# Autodesk Inventor assembly: base frame
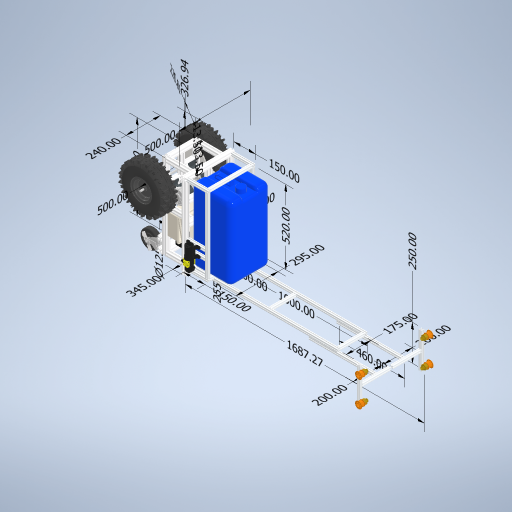
[picture p0: Inventor's stored thumbnail of the model, 512x512]
Saved by Autodesk Inventor 2023 (Build 270158000, 158)
## iProperties
Created: 2023-09-20
Part Number: base frame
Document SubType Name: Assembly
Designer: sigit
Author: sigit
## Documents named in this file (29)
- D:\Kuliah\SEMESTER 7\Robot Semprot\Design\2nd ROBOT\Assembly\base frame.iam
- D:\Kuliah\SEMESTER 7\Robot Semprot\Design\2nd ROBOT\Part\3030 600.ipt
- D:\Kuliah\SEMESTER 7\Robot Semprot\Design\2nd ROBOT\Part\3030 180.ipt
- D:\Kuliah\SEMESTER 7\Robot Semprot\Design\2nd ROBOT\Part\shaft holder 12.ipt
- D:\Kuliah\SEMESTER 7\Robot Semprot\Design\2nd ROBOT\Assembly\roda.iam
- D:\Kuliah\SEMESTER 7\Robot Semprot\Design\2nd ROBOT\Part\poros.ipt
- D:\Kuliah\SEMESTER 7\Robot Semprot\Design\2nd ROBOT\Part\free wheel 5 inch.iam
- D:\Kuliah\SEMESTER 7\Robot Semprot\Design\2nd ROBOT\Part\3030 240.ipt
- D:\Kuliah\SEMESTER 7\Robot Semprot\Design\2nd ROBOT\Part\3030 540.ipt
- D:\Kuliah\SEMESTER 7\Robot Semprot\Design\2nd ROBOT\Part\3030 75.ipt
- D:\Kuliah\SEMESTER 7\Robot Semprot\Design\2nd ROBOT\Assembly\motor+tatakan.iam
- D:\Kuliah\SEMESTER 7\Robot Semprot\Design\2nd ROBOT\Part\3030 800.ipt
- D:\Kuliah\SEMESTER 7\Robot Semprot\Design\2nd ROBOT\Part\3030 440.ipt
- D:\Kuliah\SEMESTER 7\Robot Semprot\Design\2nd ROBOT\Part\3030 470.ipt
- D:\Kuliah\SEMESTER 7\Robot Semprot\Design\2nd ROBOT\Part\jerigenn30L.ipt
- D:\Kuliah\SEMESTER 7\Robot Semprot\Design\2nd ROBOT\Part\3030 160.ipt
- D:\Kuliah\SEMESTER 7\Robot Semprot\Design\2nd ROBOT\Assembly\wadah_jerrycan.iam
- D:\Kuliah\SEMESTER 7\Robot Semprot\Design\2nd ROBOT\Part\3030 285.ipt
- D:\Kuliah\SEMESTER 7\Robot Semprot\Design\2nd ROBOT\Part\3030 113.5.ipt
- D:\Kuliah\SEMESTER 7\Robot Semprot\Design\2nd ROBOT\Part\2020 130.ipt
- D:\Kuliah\SEMESTER 7\Robot Semprot\Design\REVISI2\Part\pompa\bomba good pump.ipt
- D:\Kuliah\SEMESTER 7\Robot Semprot\Design\2nd ROBOT\Part\2020 1000.ipt
- D:\Kuliah\SEMESTER 7\Robot Semprot\Design\2nd ROBOT\Part\2020 460.ipt
- D:\Kuliah\SEMESTER 7\Robot Semprot\Design\2nd ROBOT\Part\2020 200.ipt
- D:\Kuliah\SEMESTER 7\Robot Semprot\Design\2nd ROBOT\Part\2020 250.ipt
- D:\Kuliah\SEMESTER 7\Robot Semprot\Design\2nd ROBOT\Part\2020 175.ipt
- D:\Kuliah\SEMESTER 7\Robot Semprot\Design\2nd ROBOT\Part\Junction Box Assembly.iam
- D:\Kuliah\SEMESTER 7\Robot Semprot\Design\REVISI2\Part\aki\Assembly Inventor\Aki GS GTZ5S.iam
- D:\Kuliah\SEMESTER 7\Robot Semprot\Design\REVISI2\Assembly\nozz.iam
## Components (68 placed, 28 different names)
1. 3030 600:1 — Rotational:1, Rotational:2, Rotational:9, Rotational:10, Rotational:14, Rotational:16, Rotational:18
2. 3030 600:2 — Rotational:3, Rotational:4, Rotational:11, Rotational:17, Rotational:23, Rotational:24
3. 3030 180:1 — Rotational:1, Rotational:3, Rotational:15
4. 3030 180:2 — Rotational:2
5. roda:1 [sub-assembly] — Rotational:6
6. poros:1 — Rotational:5
7. roda:2 [sub-assembly] — Rotational:7
8. free wheel 5 inch:1 [sub-assembly] — Rigid:1
9. free wheel 5 inch:2 [sub-assembly] — Rigid:2
10. 3030 180:4 — Rotational:9
11. 3030 180:5 — Rotational:10
12. 3030 180:6 — Rotational:14
13. 3030 540:1 — Rotational:15, Rotational:19, Rotational:38
14. 3030 75:1 — Rotational:16
15. 3030 75:2 — Rotational:17
16. motor+tatakan:1 [sub-assembly] — Rotational:18
17. motor+tatakan:2 [sub-assembly] — Rotational:19
18. jerigenn30L:1 — Rigid:3
19. wadah_jerrycan:1 [sub-assembly] — Rotational:25, Rotational:28, Rotational:31
20. jerigenn30L:2 — Rigid:4
21. bomba good pump:1 — Rotational:29
22. bomba good pump:2 — Rotational:30
23. 2020 200:1 — Rotational:33, Rotational:35
24. 2020 200:2 — Rotational:34, Rotational:36
25. 2020 250:1 — Rotational:35, Rigid:7
26. 2020 250:2 — Rotational:36, Rigid:6
27. Junction Box Assembly:1 [sub-assembly] — Rigid:5
28. Aki GS GTZ5S:1 [sub-assembly] — Rotational:38, Rigid:5
29. shaft holder 12:1 — Rotational:4, Rotational:5, Rotational:7
30. shaft holder 12:2 — Rotational:6
31. 3030 240:1 — Rotational:11, Rigid:1, Rigid:2
32. 3030 240:2
33. 3030 800:1 — Rotational:21
34. 3030 800:2
35. 3030 470:1 — Rotational:22
36. 3030 470:2
37. 3030 160:5 — Rotational:24, Rotational:26
38. 3030 160:6
39. 3030 285:2 — Rotational:26, Rigid:4
40. 3030 285:3 — Rotational:27
41. 3030 113.5:1 — Rotational:27
42. 3030 113.5:2
43. 2020 460:1 — Rotational:32, Rotational:33
44. 2020 1000:1 — Rotational:31, Rotational:32
45. 2020 460:2 — Rotational:34
46. 2020 1000:2 — Rotational:37
47. 2020 175:1 — Rotational:37
48. 2020 175:2
49. nozz:2 [sub-assembly] — Rigid:7
50. nozz:3 [sub-assembly]
51. nozz:4 [sub-assembly]
52. nozz:5 [sub-assembly]
53. nozz:1 [sub-assembly] — Rigid:6
54. nozz:6 [sub-assembly]
55. nozz:7 [sub-assembly]
56. nozz:8 [sub-assembly]
57. 3030 440:1 — Rotational:21
58. 3030 440:2
59. 3030 440:3
60. 3030 440:4 — Rotational:22, Rigid:3
61. 3030 160:1 — Rotational:23
62. 3030 160:2
63. 3030 160:3
64. 3030 160:4 — Rotational:25
65. 2020 130:1 — Rotational:28, Rotational:29
66. 2020 130:2
67. 2020 130:3
68. 2020 130:4 — Rotational:30
## Component patterns: (2 elements, first: shaft holder 12:1), (2 elements, first: 3030 240:1), (2 elements, first: 3030 800:1), (2 elements), (2 elements, first: 3030 470:1), (2 elements), (2 elements, first: 3030 160:5), (2 elements, first: 3030 285:2), (2 elements, first: 3030 113.5:1), (2 elements), (2 elements, first: 2020 460:1 + 2020 1000:1), (2 elements, first: 2020 175:1), (4 elements, first: nozz:2), (4 elements, first: nozz:1), (2 elements, first: 3030 440:1), Component Pattern 11:2 (2 elements), (2 elements, first: 3030 160:1), Component Pattern 14:2 (2 elements), (2 elements, first: 2020 130:1), Component Pattern 21:2 (2 elements)
## Relationships (42: RevoluteJoint 34, WeldJoint 7, Flush 1)
- Rotational:1 [RevoluteJoint] (9.486 mm): 3030 600:1 ↔ 3030 180:1
- Rotational:2 [RevoluteJoint] (9.486 mm): 3030 600:1 ↔ 3030 180:2
- Rotational:3 [RevoluteJoint] (9.486 mm): 3030 600:2 ↔ 3030 180:1
- Rotational:4 [RevoluteJoint] (9.486 mm): 3030 600:2 ↔ shaft holder 12:1
- Rotational:5 [RevoluteJoint] (362 mm): poros:1 ↔ shaft holder 12:1
- Rotational:6 [RevoluteJoint] (-20 mm): roda:1 ↔ shaft holder 12:2
- Rotational:7 [RevoluteJoint] (-20 mm): roda:2 ↔ shaft holder 12:1
- Rotational:9 [RevoluteJoint] (9.486 mm): 3030 600:1 ↔ 3030 180:4
- Rotational:10 [RevoluteJoint] (9.486 mm): 3030 600:1 ↔ 3030 180:5
- Rotational:11 [RevoluteJoint] (18.972 mm): 3030 600:2 ↔ 3030 240:1
- Rigid:1 [WeldJoint]: free wheel 5 inch:1 ↔ 3030 240:1
- Rigid:2 [WeldJoint]: free wheel 5 inch:2 ↔ 3030 240:1
- Rotational:14 [RevoluteJoint] (9.486 mm): 3030 600:1 ↔ 3030 180:6
- Rotational:15 [RevoluteJoint] (9.486 mm): 3030 180:1 ↔ 3030 540:1
- Rotational:16 [RevoluteJoint] (9.486 mm): 3030 600:1 ↔ 3030 75:1
- Rotational:17 [RevoluteJoint] (9.486 mm): 3030 600:2 ↔ 3030 75:2
- Rotational:18 [RevoluteJoint] (9.486 mm): 3030 600:1 ↔ motor+tatakan:1
- Rotational:19 [RevoluteJoint] (9.486 mm): 3030 540:1 ↔ motor+tatakan:2
- Rotational:21 [RevoluteJoint] (9.486 mm): 3030 800:1 ↔ 3030 440:1
- Rotational:22 [RevoluteJoint] (9.486 mm): 3030 470:1 ↔ 3030 440:4
- Rigid:3 [WeldJoint]: jerigenn30L:1 ↔ 3030 440:4
- Rotational:23 [RevoluteJoint] (9.486 mm): 3030 600:2 ↔ 3030 160:1
- Rotational:24 [RevoluteJoint] (9.486 mm): 3030 600:2 ↔ 3030 160:5
- Rotational:25 [RevoluteJoint] (9.486 mm): wadah_jerrycan:1 ↔ 3030 160:4
- Rotational:26 [RevoluteJoint] (9.486 mm): 3030 160:5 ↔ 3030 285:2
- Rotational:27 [RevoluteJoint] (9.486 mm): 3030 285:3 ↔ 3030 113.5:1
- Flush:1 (192 mm)
- Rigid:4 [WeldJoint]: jerigenn30L:2 ↔ 3030 285:2
- Rotational:28 [RevoluteJoint] (6.1 mm): wadah_jerrycan:1 ↔ 2020 130:1
- Rotational:29 [RevoluteJoint] (6.1 mm): bomba good pump:1 ↔ 2020 130:1
- Rotational:30 [RevoluteJoint] (6.1 mm): bomba good pump:2 ↔ 2020 130:4
- Rotational:31 [RevoluteJoint] (9.486 mm): wadah_jerrycan:1 ↔ 2020 1000:1
- Rotational:32 [RevoluteJoint] (12.2 mm): 2020 460:1 ↔ 2020 1000:1
- Rotational:33 [RevoluteJoint] (-6.1 mm): 2020 200:1 ↔ 2020 460:1
- Rotational:34 [RevoluteJoint] (-6.1 mm): 2020 200:2 ↔ 2020 460:2
- Rotational:35 [RevoluteJoint] (-6.1 mm): 2020 200:1 ↔ 2020 250:1
- Rotational:36 [RevoluteJoint] (-6.1 mm): 2020 200:2 ↔ 2020 250:2
- Rotational:37 [RevoluteJoint] (6.1 mm): 2020 1000:2 ↔ 2020 175:1
- Rotational:38 [RevoluteJoint] (9.486 mm): 3030 540:1 ↔ Aki GS GTZ5S:1
- Rigid:5 [WeldJoint] (12 mm): Junction Box Assembly:1 ↔ Aki GS GTZ5S:1
- Rigid:6 [WeldJoint]: 2020 250:2 ↔ nozz:1
- Rigid:7 [WeldJoint]: 2020 250:1 ↔ nozz:2
